# Autodesk Inventor assembly: KJ110FT33×°ÅäÌå
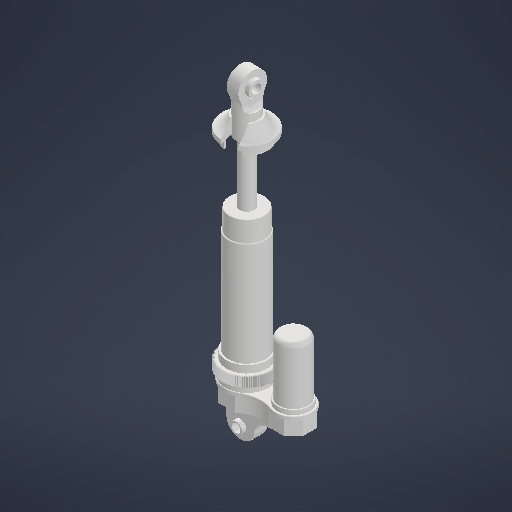
[picture p0: Inventor's stored thumbnail of the model, 512x512]
Saved by Autodesk Inventor 2025 (Build 290162000, 162)
## iProperties
Company: Î¢ÈíÖÐ¹ú
Created: 2019-03-11
Part Number: KJ110FT33×°ÅäÌå
Description: STEP AP203
Document SubType Name: Assembly
Designer: XH
Sending System: SolidWorks 2016
Preprocessor: SwSTEP 2.0
Title: KJ110FT33×°ÅäÌå.STEP
Author: Î¢ÈíÓÃ»§
Revision Number: ÈÎºÎ
## Documents named in this file (5)
- C:\1A_Engineering_files\月球车\KJ110FT33装配体.iam
- C:\1A_Engineering_files\月球车\KJ110FT33µ¯»É.ipt
- C:\1A_Engineering_files\月球车\KJ110FT33¶Ë¸Ç.ipt
- C:\1A_Engineering_files\月球车\KJ110FT33¶ËÍ·.ipt
- C:\1A_Engineering_files\月球车\KJ110FT33¿ò¼Ü.ipt
## Components (4 placed, 4 different names)
1. KJ110FT33µ¯»É_1
2. KJ110FT33¶Ë¸Ç_2 — 配合:2
3. KJ110FT33¶ËÍ·_3 — 配合:3
4. KJ110FT33¿ò¼Ü_4 — 配合:2, 配合:3
## Relationships (2: Mate 2)
- 配合:2 [Mate]: KJ110FT33¶Ë¸Ç_2 ↔ KJ110FT33¿ò¼Ü_4
- 配合:3 [Mate]: KJ110FT33¶ËÍ·_3 ↔ KJ110FT33¿ò¼Ü_4
